# Autodesk Inventor assembly: Hand Kwik-Mount
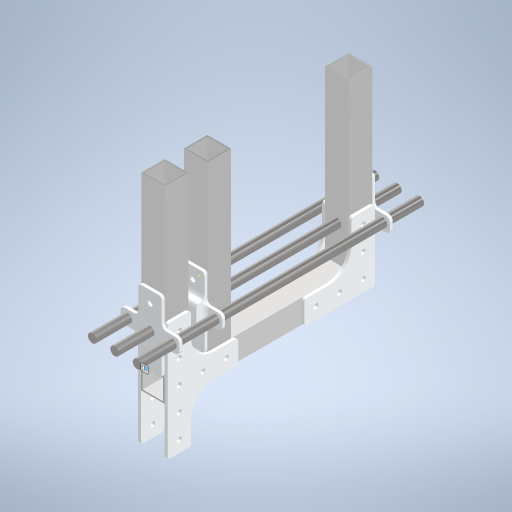
[picture p0: Inventor's stored thumbnail of the model, 512x512]
Saved by Autodesk Inventor 2024 (Build 280153000, 153)
## iProperties
Created: 2024-01-20
Part Number: Hand Kwik-Mount
Document SubType Name: Assembly
Designer: aidan
Author: aidan
## Documents named in this file (8)
- C:\Users\aidan\OneDrive\Documents\Inventor\Content Center Files\Hand Kwik-Mount.iam
- C:\Users\aidan\OneDrive\Documents\Inventor\Content Center Files\am-4158 1IN Tee Gusset.ipt
- C:\Users\aidan\OneDrive\Documents\Inventor\Content Center Files\am-3860 90 Gusset REV2.ipt
- C:\Users\aidan\OneDrive\Documents\Inventor\Content Center Files\Tube Finger.ipt
- C:\Users\aidan\OneDrive\Documents\Inventor\Content Center Files\Lead Nut Holder Mk2.ipt
- C:\Users\aidan\OneDrive\Documents\Inventor\Content Center Files\Guide Rod Holder.ipt
- C:\Users\aidan\OneDrive\Documents\Inventor\Content Center Files\Finger Base.ipt
- C:\Users\aidan\OneDrive\Documents\Inventor\Content Center Files\Lead_Shaft.ipt
## Components (14 placed, 7 different names)
1. am-3860 90 Gusset REV2:1
2. am-3860 90 Gusset REV2:2 — Rotational:4
3. Tube Finger:1 — Mate:1, Rotational:3
4. Tube Finger:2 — Mate:1
5. Lead Nut Holder Mk2:1
6. Tube Finger:3 — Rotational:7
7. Guide Rod Holder:1 — Rotational:3
8. Finger Base:1 — Rotational:4, Rotational:5, Rotational:6
9. am-4158 1IN Tee Gusset:1 — Rotational:6
10. am-4158 1IN Tee Gusset:2 — Rotational:5
11. Guide Rod Holder:2 — Rotational:7, Rotational:8, Rotational:9, Rotational:10
12. Lead_Shaft:1 — Rotational:10
13. Lead_Shaft:2 — Rotational:9
14. Lead_Shaft:3 — Rotational:8
## Relationships (9: RevoluteJoint 8, Mate 1)
- Mate:1 (127 mm): Tube Finger:1 ↔ Tube Finger:2
- Rotational:3 [RevoluteJoint]: Tube Finger:1 ↔ Guide Rod Holder:1
- Rotational:4 [RevoluteJoint]: am-3860 90 Gusset REV2:2 ↔ Finger Base:1
- Rotational:5 [RevoluteJoint]: Finger Base:1 ↔ am-4158 1IN Tee Gusset:2
- Rotational:6 [RevoluteJoint]: Finger Base:1 ↔ am-4158 1IN Tee Gusset:1
- Rotational:7 [RevoluteJoint]: Tube Finger:3 ↔ Guide Rod Holder:2
- Rotational:8 [RevoluteJoint] (-38.1 mm): Guide Rod Holder:2 ↔ Lead_Shaft:3
- Rotational:9 [RevoluteJoint] (-38.1 mm): Guide Rod Holder:2 ↔ Lead_Shaft:2
- Rotational:10 [RevoluteJoint] (-38.1 mm): Guide Rod Holder:2 ↔ Lead_Shaft:1
